# Autodesk Inventor assembly: simulink
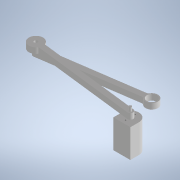
[picture p0: Inventor's stored thumbnail of the model, 180x180]
Saved by Autodesk Inventor 2021 (Build 250183000, 183)
## iProperties
Created: 2022-10-24
Part Number: simulink
Document SubType Name: Assembly
Designer: ivanm
Author: ivanm
## Documents named in this file (4)
- C:\Users\ivanm\OneDrive\Servomecanismos\Proyectos\Proyecto academico\Servomecanismo2R\INVENTOR\simulink.iam
- C:\Users\ivanm\OneDrive\Servomecanismos\Proyectos\Proyecto academico\Servomecanismo2R\INVENTOR\bancada.ipt
- C:\Users\ivanm\OneDrive\Servomecanismos\Proyectos\Proyecto academico\Servomecanismo2R\INVENTOR\eslabon1.ipt
- C:\Users\ivanm\OneDrive\Servomecanismos\Proyectos\Proyecto academico\Servomecanismo2R\INVENTOR\eslabon2.ipt
## Components (3 placed, 3 different names)
1. bancada:1 — De rotación:1
2. eslabon1:1 — De rotación:1, De rotación:2
3. eslabon2:1 — De rotación:2
## Relationships (2: RevoluteJoint 2)
- De rotación:1 [RevoluteJoint]: bancada:1 ↔ eslabon1:1
- De rotación:2 [RevoluteJoint]: eslabon1:1 ↔ eslabon2:1
